# Autodesk Inventor assembly: 4_WheelsSwerve01
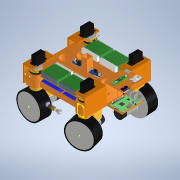
[picture p0: Inventor's stored thumbnail of the model, 180x180]
Saved by Autodesk Inventor 2021 (Build 250183000, 183)
## iProperties
Created: 2021-11-14
Part Number: 4_WheelsSwerve01
Document SubType Name: Assembly
Designer: techv
Sending System: Autodesk Translation Framework v10.10.0.1391
Preprocessor: ST-DEVELOPER v18.1
Title: c:\worker\convert-fusion-r08\tmp\job-1\18\output\files\00ab14de-8d8f-4ea9-b8db-e980fd0b2348\42fddb95-f990-4b6e-b7ef-776fa718d36f.stp
## Documents named in this file (24)
- D:\Projects\P_Intelligent Line Marking Bot\Design\3D cad xrobot version\OnmiSwerve-main\CAD\4_WheelsSwerve01.iam
- D:\Projects\P_Intelligent Line Marking Bot\Design\3D cad xrobot version\OnmiSwerve-main\CAD\wheel.ipt
- D:\Projects\P_Intelligent Line Marking Bot\Design\3D cad xrobot version\OnmiSwerve-main\CAD\wheel(Mirror).ipt
- D:\Projects\P_Intelligent Line Marking Bot\Design\3D cad xrobot version\OnmiSwerve-main\CAD\wheel(Mirror) (1).ipt
- D:\Projects\P_Intelligent Line Marking Bot\Design\3D cad xrobot version\OnmiSwerve-main\CAD\wheel(Mirror)(Mirror).ipt
- D:\Projects\P_Intelligent Line Marking Bot\Design\3D cad xrobot version\OnmiSwerve-main\CAD\Part10.ipt
- D:\Projects\P_Intelligent Line Marking Bot\Design\LMBOT V3 80%\Golden part.ipt
- D:\Projects\P_Intelligent Line Marking Bot\Design\LMBOT V3 80%\Part13.ipt
- D:\Projects\P_Intelligent Line Marking Bot\Design\3D cad xrobot version\my designs\servo_mount.ipt
- D:\Projects\P_Intelligent Line Marking Bot\Design\3D cad xrobot version\my designs\servo_mount_MIR.ipt
- D:\Projects\P_Intelligent Line Marking Bot\Design\LMBOT V3 80%\wheel_MIR_MIR.ipt
- D:\Projects\A_Electronics CAD model\raspberry-pi-27.snapshot.7\RaspberryPi.iam
- D:\Projects\A_Electronics CAD model\ublox-gps-1.snapshot.1\gps\parts\GPS_ublox_board.ipt
- C:\Users\techv\Documents\Teensy.ipt
- C:\Users\techv\Downloads\Teensy 4.1_TOP.iam
- D:\Projects\A_Electronics CAD model\mpu-9250-9dof-imu-1.snapshot.4\MPU-9250.iam
- C:\Users\techv\Documents\HCM5883L.ipt
- C:\Users\techv\Documents\C drive Inventor Files\motor driver.ipt
- D:\Projects\P_Intelligent Line Marking Bot\Design\3D cad xrobot version\my designs\battery.ipt
- C:\Users\techv\Downloads\LM2596 DC-DC StepDown Converter v1.iam
- D:\Projects\P_Intelligent Line Marking Bot\Design\3D cad xrobot version\my designs\servo flange.ipt
- D:\Projects\P_Intelligent Line Marking Bot\Design\LMBOT V3 80%\n20 geared motor.ipt
- D:\Projects\P_Intelligent Line Marking Bot\Design\LMBOT V3 80%\8mm flange nut.ipt
- D:\Projects\P_Intelligent Line Marking Bot\Design\LMBOT V3 80%\M6-lead screw.ipt
## Components (42 placed, 23 different names)
1. wheel:1 — Mate:4, Mate:22, Mate:42, Mate:48, Mate:49, Mate:86, Mate:87, Mate:88
2. wheel(Mirror):1 — Mate:1, Mate:19, Mate:43, Mate:50, Mate:51, Mate:89, Mate:90, Mate:91
3. wheel(Mirror) (1):1 — Mate:3, Mate:21, Mate:28, Mate:72, Mate:73, Mate:83, Mate:84, Mate:85
4. wheel(Mirror)(Mirror):1 — Mate:2, Mate:20, Mate:41, Mate:44, Mate:45, Flush:34
5. Part10 — Mate:1, Mate:2, Mate:3, Mate:4, Mate:19, Mate:20, Mate:21, Mate:22, Mate:23, Mate:24, Mate:25, Mate:26, Flush:1, Mate:27, Angle:1, Mate:30, Flush:2, Mate:31, Flush:3, Mate:35, Mate:36, Mate:37, Mate:38, Mate:39, Mate:40, Angle:2, Angle:3, Angle:4, Mate:52, Mate:61, Flush:15, Flush:16, Mate:62, Flush:17, Mate:63, Flush:18, Mate:64, Mate:65, Flush:21, Flush:22, Mate:67, Flush:23, Flush:24, Mate:68, Flush:25, Mate:69, Flush:26, Flush:27, Mate:70, Mate:71, Flush:28, Flush:29, Flush:30, Mate:74, Mate:75, Mate:76, Mate:77, Mate:78, Mate:79, Mate:80, Flush:31, Flush:32, Mate:81, Flush:33
6. Golden part:1 — Mate:9, Mate:10, Mate:28
7. Part13:1 — Mate:9, Mate:10, Mate:29, Angle:1
8. Golden part:2
9. Part13:2 — Mate:32, Mate:43, Angle:2
10. Golden part:3
11. Part13:3 — Mate:34, Mate:42, Angle:3
12. Golden part:4
13. Part13:4 — Mate:33, Mate:41, Angle:4
14. servo_mount:1 — Mate:26, Flush:1, Mate:27, Mate:29
15. servo_mount:2 — Mate:30, Flush:2, Mate:31, Mate:33
16. servo_mount_MIR:1 — Mate:32, Mate:38, Mate:39, Mate:40
17. servo_mount_MIR:2 — Mate:34, Mate:35, Mate:36, Mate:37
18. wheel_MIR_MIR:1 — Mate:44, Mate:45
19. wheel_MIR_MIR:2 — Mate:48, Mate:49
20. wheel_MIR_MIR:3 — Mate:50, Mate:51
21. wheel_MIR_MIR:4 — Mate:72, Mate:73
22. RaspberryPi:1 [sub-assembly] — Mate:52, Flush:28, Flush:29
23. GPS_ublox_board:1 — Flush:21, Flush:22, Mate:67
24. Teensy:1
25. MPU-9250:2 [sub-assembly] — Flush:27, Mate:70, Mate:71
26. Teensy 4.1_TOP:2 [sub-assembly] — Flush:25, Mate:69, Flush:26
27. HCM5883L:1 — Flush:23, Flush:24, Mate:68
28. motor driver:1 — Mate:61, Flush:15, Mate:66, Flush:19
29. motor driver:2 — Flush:18, Mate:64, Flush:20
30. motor driver:3 — Flush:16, Mate:62, Mate:65, Mate:66, Flush:20
31. motor driver:4 — Flush:17, Mate:63, Flush:19
32. battery:1 — Flush:30, Mate:74, Mate:75, Mate:76
33. battery:2 — Mate:77, Mate:78, Mate:79
34. LM2596 DC-DC StepDown Converter v1:1 [sub-assembly] — Mate:80, Flush:31, Flush:32, Mate:82
35. LM2596 DC-DC StepDown Converter v1:2 [sub-assembly] — Mate:81, Flush:33, Mate:82
36. servo flange:1 — Flush:34
37. servo flange:2 — Mate:89, Mate:90, Mate:91
38. servo flange:3 — Mate:86, Mate:87, Mate:88
39. servo flange:4 — Mate:83, Mate:84, Mate:85
40. n20 geared motor:1 — Mate:93
41. 8mm flange nut:1 — Mate:92
42. M6-lead screw:1 — Mate:92, Mate:93
## Relationships (104: Mate 77, Flush 23, Angle 4)
- Mate:1: wheel(Mirror):1 ↔ Part10
- Mate:2: wheel(Mirror)(Mirror):1 ↔ Part10
- Mate:3: wheel(Mirror) (1):1 ↔ Part10
- Mate:4: wheel:1 ↔ Part10
- Mate:9: Golden part:1 ↔ Part13:1
- Mate:10: Golden part:1 ↔ Part13:1
- [Mate]: Golden part:2 ↔ Part13:2
- [Mate]: Golden part:2 ↔ Part13:2
- [Mate]: Golden part:3 ↔ Part13:3
- [Mate]: Golden part:3 ↔ Part13:3
- [Mate]: Golden part:4 ↔ Part13:4
- [Mate]: Golden part:4 ↔ Part13:4
- Mate:19: wheel(Mirror):1 ↔ Part10
- Mate:20: wheel(Mirror)(Mirror):1 ↔ Part10
- Mate:21: wheel(Mirror) (1):1 ↔ Part10
- Mate:22: wheel:1 ↔ Part10
- Mate:23: Part10
- Mate:24: Part10
- Mate:25: Part10
- Mate:26: Part10 ↔ servo_mount:1
- Flush:1: Part10 ↔ servo_mount:1
- Mate:27: Part10 ↔ servo_mount:1
- Mate:28: wheel(Mirror) (1):1 ↔ Golden part:1
- Mate:29: Part13:1 ↔ servo_mount:1
- Angle:1 (0 deg): Part10 ↔ Part13:1
- Mate:30: Part10 ↔ servo_mount:2
- Flush:2: Part10 ↔ servo_mount:2
- Mate:31: Part10 ↔ servo_mount:2
- Flush:3 (-141.25 mm): Part10
- Mate:32: Part13:2 ↔ servo_mount_MIR:1
- Mate:33: Part13:4 ↔ servo_mount:2
- Mate:34: Part13:3 ↔ servo_mount_MIR:2
- Mate:35: Part10 ↔ servo_mount_MIR:2
- Mate:36: Part10 ↔ servo_mount_MIR:2
- Mate:37: Part10 ↔ servo_mount_MIR:2
- Mate:38: Part10 ↔ servo_mount_MIR:1
- Mate:39: Part10 ↔ servo_mount_MIR:1
- Mate:40: Part10 ↔ servo_mount_MIR:1
- Mate:41: wheel(Mirror)(Mirror):1 ↔ Part13:4
- Mate:42: wheel:1 ↔ Part13:3
- Mate:43: wheel(Mirror):1 ↔ Part13:2
- Angle:2 (0 deg): Part10 ↔ Part13:2
- Angle:3 (0 deg): Part10 ↔ Part13:3
- Angle:4 (0 deg): Part10 ↔ Part13:4
- Mate:44: wheel(Mirror)(Mirror):1 ↔ wheel_MIR_MIR:1
- Mate:45: wheel(Mirror)(Mirror):1 ↔ wheel_MIR_MIR:1
- Mate:48: wheel:1 ↔ wheel_MIR_MIR:2
- Mate:49: wheel:1 ↔ wheel_MIR_MIR:2
- Mate:50: wheel(Mirror):1 ↔ wheel_MIR_MIR:3
- Mate:51: wheel(Mirror):1 ↔ wheel_MIR_MIR:3
- Mate:52: Part10 ↔ RaspberryPi:1
- Mate:61: Part10 ↔ motor driver:1
- Flush:15: Part10 ↔ motor driver:1
- Flush:16: Part10 ↔ motor driver:3
- Mate:62: Part10 ↔ motor driver:3
- Flush:17: Part10 ↔ motor driver:4
- Mate:63: Part10 ↔ motor driver:4
- Flush:18: Part10 ↔ motor driver:2
- Mate:64: Part10 ↔ motor driver:2
- Mate:65 (10 mm): Part10 ↔ motor driver:3
- Mate:66 (10 mm): motor driver:1 ↔ motor driver:3
- Flush:19: motor driver:1 ↔ motor driver:4
- Flush:20: motor driver:2 ↔ motor driver:3
- Flush:21 (3 mm): Part10 ↔ GPS_ublox_board:1
- Flush:22 (3 mm): Part10 ↔ GPS_ublox_board:1
- Mate:67 (3 mm): Part10 ↔ GPS_ublox_board:1
- Flush:23 (3 mm): Part10 ↔ HCM5883L:1
- Flush:24 (3 mm): Part10 ↔ HCM5883L:1
- Mate:68 (3 mm): Part10 ↔ HCM5883L:1
- Flush:25 (3 mm): Part10 ↔ Teensy 4.1_TOP:2
- Mate:69 (3 mm): Part10 ↔ Teensy 4.1_TOP:2
- Flush:26 (20 mm): Part10 ↔ Teensy 4.1_TOP:2
- Flush:27 (3 mm): Part10 ↔ MPU-9250:2
- Mate:70 (3 mm): Part10 ↔ MPU-9250:2
- Mate:71 (1.5 mm): Part10 ↔ MPU-9250:2
- Flush:28 (3 mm): Part10 ↔ RaspberryPi:1
- Flush:29 (6 mm): Part10 ↔ RaspberryPi:1
- Mate:72: wheel(Mirror) (1):1 ↔ wheel_MIR_MIR:4
- Mate:73: wheel(Mirror) (1):1 ↔ wheel_MIR_MIR:4
- Flush:30: Part10 ↔ battery:1
- Mate:74: Part10 ↔ battery:1
- Mate:75: Part10 ↔ battery:1
- Mate:76: Part10 ↔ battery:1
- Mate:77: Part10 ↔ battery:2
- Mate:78: Part10 ↔ battery:2
- Mate:79: Part10 ↔ battery:2
- Mate:80 (3 mm): Part10 ↔ LM2596 DC-DC StepDown Converter v1:1
- Flush:31 (70 mm): Part10 ↔ LM2596 DC-DC StepDown Converter v1:1
- Flush:32 (15 mm): Part10 ↔ LM2596 DC-DC StepDown Converter v1:1
- Mate:81 (3 mm): Part10 ↔ LM2596 DC-DC StepDown Converter v1:2
- Flush:33 (15 mm): Part10 ↔ LM2596 DC-DC StepDown Converter v1:2
- Mate:82 (30 mm): LM2596 DC-DC StepDown Converter v1:1 ↔ LM2596 DC-DC StepDown Converter v1:2
- Flush:34: wheel(Mirror)(Mirror):1 ↔ servo flange:1
- Mate:83: wheel(Mirror) (1):1 ↔ servo flange:4
- Mate:84: wheel(Mirror) (1):1 ↔ servo flange:4
- Mate:85: wheel(Mirror) (1):1 ↔ servo flange:4
- Mate:86: wheel:1 ↔ servo flange:3
- Mate:87: wheel:1 ↔ servo flange:3
- Mate:88: wheel:1 ↔ servo flange:3
- Mate:89: wheel(Mirror):1 ↔ servo flange:2
- Mate:90: wheel(Mirror):1 ↔ servo flange:2
- Mate:91: wheel(Mirror):1 ↔ servo flange:2
- Mate:92: 8mm flange nut:1 ↔ M6-lead screw:1
- Mate:93: n20 geared motor:1 ↔ M6-lead screw:1
## Named parameters: d10_d9 = 0 mm, d11_d8 = 0 mm, d12_d9 = 0 mm, d13_d8 = 0 mm, d14_d9 = 0 mm, d15_d8 = 0 mm
